# Autodesk Inventor assembly: x axys
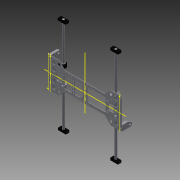
[picture p0: Inventor's stored thumbnail of the model, 180x180]
Saved by Autodesk Inventor 2014 SP1 (Build 180222100, 222)
## iProperties
Created: 2015-04-08
Part Number: x axys
Document SubType Name: Assembly
Designer: Giorgio Nuzzo
Author: Giorgio Nuzzo
## Documents named in this file (19)
- C:\Users\Giorgio Nuzzo\Desktop\3dragmodel\x axys.iam
- C:\Users\Giorgio Nuzzo\Desktop\3dragmodel\supporto_manicotto_X.ipt
- C:\Users\Giorgio Nuzzo\Desktop\3dragmodel\cuscinetto_X.ipt
- C:\Users\Giorgio Nuzzo\Desktop\3dragmodel\piastraX.ipt
- C:\Users\Giorgio Nuzzo\Desktop\3dragmodel\supporto_manicotto_X_MIR.ipt
- C:\Users\Giorgio Nuzzo\Desktop\3dragmodel\cuscinetto_X_MIR.ipt
- C:\Users\Giorgio Nuzzo\Desktop\3dragmodel\supporto_manicotto_X_MIR1.ipt
- C:\Users\Giorgio Nuzzo\Desktop\3dragmodel\cuscinetto_X_MIR1.ipt
- C:\Users\Giorgio Nuzzo\Desktop\3dragmodel\supporto_manicotto_X_MIR_MIR.ipt
- C:\Users\Giorgio Nuzzo\Desktop\3dragmodel\cuscinetto_X_MIR_MIR.ipt
- C:\Users\Giorgio Nuzzo\Desktop\3dragmodel\barra X.ipt
- C:\Users\Giorgio Nuzzo\Desktop\3dragmodel\barra X_MIR.ipt
- C:\Users\Giorgio Nuzzo\Desktop\3dragmodel\supporto guide x.ipt
- C:\Users\Giorgio Nuzzo\Desktop\3dragmodel\supporto guide x_MIR.ipt
- C:\Users\Giorgio Nuzzo\Desktop\3dragmodel\supporto guide x_MIR1.ipt
- C:\Users\Giorgio Nuzzo\Desktop\3dragmodel\supporto guide x_MIR_MIR.ipt
- C:\Users\Giorgio Nuzzo\Desktop\3dragmodel\supporto_guide_lungo.ipt
- C:\Users\Giorgio Nuzzo\Desktop\3dragmodel\supporto_guide_corto.ipt
- C:\Users\Giorgio Nuzzo\Desktop\3dragmodel\supporto_guide_corto_MIR1.ipt
## Components (18 placed, 18 different names)
1. supporto_manicotto_X:1
2. cuscinetto_X:1
3. piastraX:1 — Flush:1, Angle:1, Flush:5, Flush:6
4. supporto_manicotto_X_MIR:1
5. cuscinetto_X_MIR:1
6. supporto_manicotto_X_MIR1:1
7. cuscinetto_X_MIR1:1
8. supporto_manicotto_X_MIR_MIR:1
9. cuscinetto_X_MIR_MIR:1
10. barra X:1 — Flush:1, Insert:1
11. barra X_MIR:1
12. supporto guide x:1 — Insert:1, Angle:1
13. supporto guide x_MIR:1
14. supporto guide x_MIR1:1
15. supporto guide x_MIR_MIR:1
16. supporto_guide_lungo:1 — Mate:2, Flush:6
17. supporto_guide_corto:1 — Mate:2, Flush:5
18. supporto_guide_corto_MIR1:1
## Relationships (6: Flush 3, Insert 1, Angle 1, Mate 1)
- Flush:1: piastraX:1 ↔ barra X:1
- Insert:1: barra X:1 ↔ supporto guide x:1
- Angle:1 (0 deg): piastraX:1 ↔ supporto guide x:1
- Mate:2: supporto_guide_lungo:1 ↔ supporto_guide_corto:1
- Flush:5: piastraX:1 ↔ supporto_guide_corto:1
- Flush:6: piastraX:1 ↔ supporto_guide_lungo:1
